# Autodesk Inventor assembly: TS_Magazin_gesamt_int
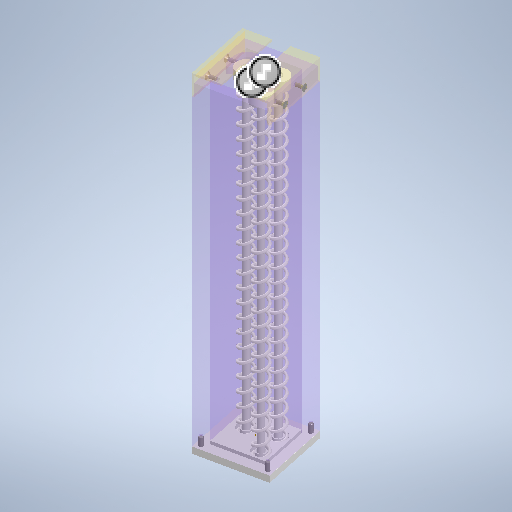
[picture p0: Inventor's stored thumbnail of the model, 512x512]
Saved by Autodesk Inventor 2025.2 (Build 292293000, 293)
## iProperties
Created: 2025-06-01
Part Number: TS_Magazin_gesamt_int
Document SubType Name: Assembly
Designer: tino
Author: tino
## Documents named in this file (12)
- C:\Users\tino\Documents_VM\Konstruieren_CAD\Useless Box\Eigene Bauteile\TS_Magazin_gesamt_int.iam
- C:\Users\tino\Documents_VM\Konstruieren_CAD\Useless Box\Eigene Bauteile\TS_Magazin_Grundplatte_int.ipt.ipt
- C:\Users\tino\Documents_VM\Konstruieren_CAD\Useless Box\Eigene Bauteile\TS_Magazin_Gehause_int.ipt
- C:\Users\tino\Documents_VM\Konstruieren_CAD\Useless Box\Eigene Bauteile\TS_Magazin_Fuehrungselement_int.ipt
- C:\Users\tino\Documents_VM\Konstruieren_CAD\Useless Box\Eigene Bauteile\TS_Magazin_Gleitbuchse_int.ipt
- C:\Users\tino\Documents_VM\Konstruieren_CAD\Useless Box\Eigene Bauteile\TS_Magazin_Druckfeder_int.ipt
- C:\Users\tino\Documents_VM\Konstruieren_CAD\Useless Box\Eigene Bauteile\TS_Magazin_Begrenzung_int.ipt
- C:\Users\tino\Documents_VM\Inventor\Content Center Files\R2025\de-DE\ISO 4762(2)\ISO 4762 - M6 x 16ISO.ipt
- C:\Users\tino\Documents_VM\Inventor\Content Center Files\R2025\de-DE\ISO 4762(2)\ISO 4762 - M6 x 12ISO.ipt
- C:\Users\tino\Documents_VM\Inventor\Content Center Files\R2025\de-DE\DIN 7991(2)\DIN 7991 - M5x12.ipt
- C:\Users\tino\Documents_VM\Konstruieren_CAD\Useless Box\Eigene Bauteile\TS_Magazin_Begrenzung_int_MIR1.ipt
- TS_Magazin_Grundplatte_int.ipt
## Components (24 placed, 10 different names)
1. TS_Magazin_Grundplatte_int.ipt:1 — Passend:1, Passend:2, Passend:3, Passend:4, Passend:5, Passend:6, Passend:7, Passend:8, Passend:9, Fluchtend:6, Passend:19, Passend:21, Passend:26, Passend:27, Passend:28, Passend:29, Passend:30, Passend:31, Passend:32, Passend:33
2. TS_Magazin_Gehause_int:1 — Passend:7, Passend:8, Passend:9, Passend:23, Passend:24, Passend:25, Passend:34
3. TS_Magazin_Fuehrungselement_int:1 — Passend:1, Passend:6, Passend:12, Passend:17
4. TS_Magazin_Fuehrungselement_int:2 — Passend:2, Passend:5, Passend:10, Passend:20
5. TS_Magazin_Fuehrungselement_int:3 — Passend:3, Passend:4, Passend:11, Passend:22
6. TS_Magazin_Gleitbuchse_int:1 — Passend:10, Fluchtend:1
7. TS_Magazin_Gleitbuchse_int:2 — Passend:11, Fluchtend:2
8. TS_Magazin_Gleitbuchse_int:3 — Passend:12, Fluchtend:1, Fluchtend:2, Passend:18
9. Druckfeder1:1 — Passend:17, Fluchtend:6, Passend:18
10. Druckfeder1:2 — Passend:19, Passend:20
11. Druckfeder1:3 — Passend:21, Passend:22
12. TS_Magazin_Begrenzung_int:1 — Passend:23, Passend:24, Passend:25, Tangential:1, Passend:35, Tangential:2
13. ISO 4762 M6 x 12:1 — Passend:32, Passend:33
14. ISO 4762 M6 x 12:2 — Passend:30, Passend:31
15. ISO 4762 M6 x 12:3 — Passend:28, Passend:29
16. DIN 7991 M5x12:1 — Passend:35, Tangential:2
17. DIN 7991 M5x12:2 — Passend:34, Tangential:1
18. DIN 7991 M5x12:3
19. DIN 7991 M5x12:4
20. TS_Magazin_Begrenzung_int_MIR1:1
21. ISO 4762 M6 x 16:1 — Passend:26, Passend:27
22. ISO 4762 M6 x 16:2
23. ISO 4762 M6 x 16:3
24. ISO 4762 M6 x 16:4
## Component patterns: (4 elements, first: ISO 4762 M6 x 16:1)
## Relationships (36: Mate 31, Flush 3, Tangent 2)
- Passend:1 [Mate]: TS_Magazin_Grundplatte_int.ipt:1 ↔ TS_Magazin_Fuehrungselement_int:1
- Passend:2 [Mate]: TS_Magazin_Grundplatte_int.ipt:1 ↔ TS_Magazin_Fuehrungselement_int:2
- Passend:3 [Mate]: TS_Magazin_Grundplatte_int.ipt:1 ↔ TS_Magazin_Fuehrungselement_int:3
- Passend:4 [Mate]: TS_Magazin_Grundplatte_int.ipt:1 ↔ TS_Magazin_Fuehrungselement_int:3
- Passend:5 [Mate]: TS_Magazin_Grundplatte_int.ipt:1 ↔ TS_Magazin_Fuehrungselement_int:2
- Passend:6 [Mate]: TS_Magazin_Grundplatte_int.ipt:1 ↔ TS_Magazin_Fuehrungselement_int:1
- Passend:7 [Mate]: TS_Magazin_Grundplatte_int.ipt:1 ↔ TS_Magazin_Gehause_int:1
- Passend:8 [Mate]: TS_Magazin_Grundplatte_int.ipt:1 ↔ TS_Magazin_Gehause_int:1
- Passend:9 [Mate]: TS_Magazin_Grundplatte_int.ipt:1 ↔ TS_Magazin_Gehause_int:1
- Passend:10 [Mate]: TS_Magazin_Fuehrungselement_int:2 ↔ TS_Magazin_Gleitbuchse_int:1
- Passend:11 [Mate]: TS_Magazin_Fuehrungselement_int:3 ↔ TS_Magazin_Gleitbuchse_int:2
- Passend:12 [Mate]: TS_Magazin_Fuehrungselement_int:1 ↔ TS_Magazin_Gleitbuchse_int:3
- Fluchtend:1 [Flush]: TS_Magazin_Gleitbuchse_int:1 ↔ TS_Magazin_Gleitbuchse_int:3
- Fluchtend:2 [Flush]: TS_Magazin_Gleitbuchse_int:2 ↔ TS_Magazin_Gleitbuchse_int:3
- Passend:17 [Mate]: TS_Magazin_Fuehrungselement_int:1 ↔ Druckfeder1:1
- Fluchtend:6 [Flush]: TS_Magazin_Grundplatte_int.ipt:1 ↔ Druckfeder1:1
- Passend:18 [Mate]: TS_Magazin_Gleitbuchse_int:3 ↔ Druckfeder1:1
- Passend:19 [Mate]: TS_Magazin_Grundplatte_int.ipt:1 ↔ Druckfeder1:2
- Passend:20 [Mate]: TS_Magazin_Fuehrungselement_int:2 ↔ Druckfeder1:2
- Passend:21 [Mate]: TS_Magazin_Grundplatte_int.ipt:1 ↔ Druckfeder1:3
- Passend:22 [Mate]: TS_Magazin_Fuehrungselement_int:3 ↔ Druckfeder1:3
- Passend:23 [Mate]: TS_Magazin_Gehause_int:1 ↔ TS_Magazin_Begrenzung_int:1
- Passend:24 [Mate]: TS_Magazin_Gehause_int:1 ↔ TS_Magazin_Begrenzung_int:1
- Passend:25 [Mate]: TS_Magazin_Gehause_int:1 ↔ TS_Magazin_Begrenzung_int:1
- Passend:26 [Mate]: TS_Magazin_Grundplatte_int.ipt:1 ↔ ISO 4762 M6 x 16:1
- Passend:27 [Mate]: TS_Magazin_Grundplatte_int.ipt:1 ↔ ISO 4762 M6 x 16:1
- Passend:28 [Mate]: TS_Magazin_Grundplatte_int.ipt:1 ↔ ISO 4762 M6 x 12:3
- Passend:29 [Mate]: TS_Magazin_Grundplatte_int.ipt:1 ↔ ISO 4762 M6 x 12:3
- Passend:30 [Mate]: TS_Magazin_Grundplatte_int.ipt:1 ↔ ISO 4762 M6 x 12:2
- Passend:31 [Mate]: TS_Magazin_Grundplatte_int.ipt:1 ↔ ISO 4762 M6 x 12:2
- Passend:32 [Mate]: TS_Magazin_Grundplatte_int.ipt:1 ↔ ISO 4762 M6 x 12:1
- Passend:33 [Mate]: TS_Magazin_Grundplatte_int.ipt:1 ↔ ISO 4762 M6 x 12:1
- Passend:34 [Mate]: TS_Magazin_Gehause_int:1 ↔ DIN 7991 M5x12:2
- Tangential:1: TS_Magazin_Begrenzung_int:1 ↔ DIN 7991 M5x12:2
- Passend:35 [Mate]: TS_Magazin_Begrenzung_int:1 ↔ DIN 7991 M5x12:1
- Tangential:2: TS_Magazin_Begrenzung_int:1 ↔ DIN 7991 M5x12:1
